# Autodesk Inventor assembly: UpperBody
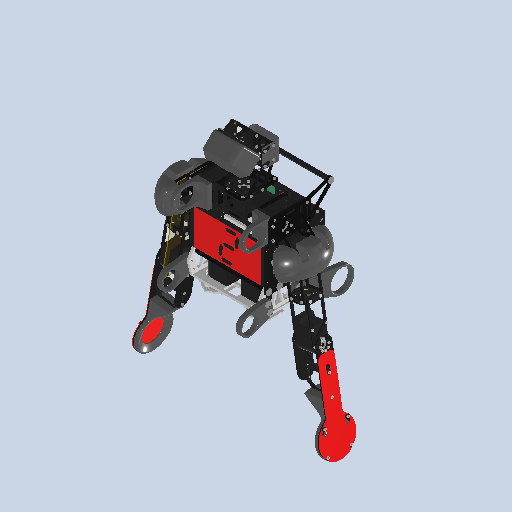
[picture p0: Inventor's stored thumbnail of the model, 512x512]
Saved by Autodesk Inventor 2022 (Build 260153000, 153)
## iProperties
Created: 2022-01-14
Part Number: UpperBody
Document SubType Name: Assembly
Designer: Masato Kubotera
Mass: 1918.95 g
Surface Area: 7006.93 cm^2
Volume: 1229.13 cm^3
Author: Masato Kubotera
## Documents named in this file (11)
- C:\Users\Masato\Documents\Inventor\CIT Brains_Inventor\SUSTAINA-OP\UpperBody\UpperBody.iam
- C:\Users\Masato\Documents\Inventor\CIT Brains_Inventor\SUSTAINA-OP\UpperBody\Trunk\Trunk.iam
- C:\Users\Masato\Documents\Inventor\CIT Brains_Inventor\SUSTAINA-OP\UpperBody\Head\Head.iam
- C:\Users\Masato\Documents\Inventor\CIT Brains_Inventor\SUSTAINA-OP\UpperBody\Arm\Shoulder.iam
- C:\Users\Masato\Documents\Inventor\CIT Brains_Inventor\SUSTAINA-OP\UpperBody\Arm\UpperArm.iam
- C:\Users\Masato\Documents\Inventor\CIT Brains_Inventor\SUSTAINA-OP\UpperBody\Arm\ForeArm.iam
- C:\Users\Masato\Documents\Inventor\CIT Brains_Inventor\SUSTAINA-OP\UpperBody\Arm\UpperArm_MIR.iam
- C:\Users\Masato\Documents\Inventor\CIT Brains_Inventor\SUSTAINA-OP\UpperBody\Cockpit\Cockpit.iam
- C:\Users\Masato\Documents\Inventor\CIT Brains_Inventor\SUSTAINA-OP\UpperBody\Arm\ForeArm_hand.ipt
- C:\Users\Masato\Documents\Inventor\CIT Brains_Inventor\SUSTAINA-OP\ReadyMade\InsertNut\UD-43040.ipt
- C:\Users\Masato\Documents\Inventor\CIT Brains_Inventor\SUSTAINA-OP\UpperBody\Arm\SideBumper.ipt
## Components (21 placed, 10 different names)
1. Trunk:1 [sub-assembly] — フラッシュ:1, フラッシュ:2, フラッシュ:3, 挿入:1, 角度:1, 挿入:2, 挿入:3, 角度:2, 角度:3, 挿入:11
2. Head:1 [sub-assembly] — 挿入:1, 角度:1
3. Shoulder:1 [sub-assembly] — 挿入:2, 角度:2, 挿入:4, 角度:4
4. Shoulder:2 [sub-assembly] — 挿入:3, 角度:3, 挿入:9, 角度:7
5. UpperArm:1 [sub-assembly] — 挿入:4, 角度:4, 挿入:6, 角度:6, フラッシュ:4, フラッシュ:5, フラッシュ:6
6. ForeArm:1 [sub-assembly] — 挿入:6, 角度:6, 挿入:20, 挿入:21
7. ForeArm:2 [sub-assembly] — 挿入:10, 角度:8, 挿入:22, 挿入:23
8. UpperArm_MIR:1 [sub-assembly] — 挿入:9, 挿入:10, 角度:7, 角度:8, メイト:1, メイト:2, フラッシュ:7
9. Cockpit:1 [sub-assembly] — 挿入:11, 角度:9
10. ForeArm_hand:1 — 挿入:12, 挿入:13, 挿入:14, 挿入:15
11. ForeArm_hand:2 — 挿入:16, 挿入:17, 挿入:18, 挿入:19
12. SideBumper:1 — フラッシュ:4, フラッシュ:5, フラッシュ:6
13. SideBumper:2 — メイト:1, メイト:2, フラッシュ:7
14. UD-43040:1 — 挿入:12, 挿入:20
15. UD-43040:2 — 挿入:13, 挿入:21
16. UD-43040:3 — 挿入:14
17. UD-43040:4 — 挿入:15
18. UD-43040:5 — 挿入:16, 挿入:23
19. UD-43040:6 — 挿入:17
20. UD-43040:7 — 挿入:18, 挿入:22
21. UD-43040:8 — 挿入:19
## Relationships (37: Insert 20, Angle 8, Flush 7, Mate 2)
- フラッシュ:1 [Flush]: Trunk:1
- フラッシュ:2 [Flush]: Trunk:1
- フラッシュ:3 [Flush]: Trunk:1
- 挿入:1 [Insert]: Trunk:1 ↔ Head:1
- 角度:1 [Angle] (0 deg): Trunk:1 ↔ Head:1
- 挿入:2 [Insert]: Trunk:1 ↔ Shoulder:1
- 挿入:3 [Insert]: Trunk:1 ↔ Shoulder:2
- 角度:2 [Angle] (0 deg): Trunk:1 ↔ Shoulder:1
- 角度:3 [Angle] (0 deg): Trunk:1 ↔ Shoulder:2
- 挿入:4 [Insert]: Shoulder:1 ↔ UpperArm:1
- 角度:4 [Angle] (170 deg): Shoulder:1 ↔ UpperArm:1
- 挿入:6 [Insert]: UpperArm:1 ↔ ForeArm:1
- 角度:6 [Angle] (0 deg): UpperArm:1 ↔ ForeArm:1
- 挿入:9 [Insert]: Shoulder:2 ↔ UpperArm_MIR:1
- 挿入:10 [Insert]: ForeArm:2 ↔ UpperArm_MIR:1
- 角度:7 [Angle] (10 deg): Shoulder:2 ↔ UpperArm_MIR:1
- 角度:8 [Angle] (180 deg): ForeArm:2 ↔ UpperArm_MIR:1
- 挿入:11 [Insert] (0.025 mm): Trunk:1 ↔ Cockpit:1
- 角度:9 [Angle] (0 deg): Cockpit:1
- 挿入:12 [Insert]: ForeArm_hand:1 ↔ UD-43040:1
- 挿入:13 [Insert]: ForeArm_hand:1 ↔ UD-43040:2
- 挿入:14 [Insert]: ForeArm_hand:1 ↔ UD-43040:3
- 挿入:15 [Insert]: ForeArm_hand:1 ↔ UD-43040:4
- 挿入:16 [Insert]: ForeArm_hand:2 ↔ UD-43040:5
- 挿入:17 [Insert]: ForeArm_hand:2 ↔ UD-43040:6
- 挿入:18 [Insert]: ForeArm_hand:2 ↔ UD-43040:7
- 挿入:19 [Insert]: ForeArm_hand:2 ↔ UD-43040:8
- 挿入:20 [Insert]: ForeArm:1 ↔ UD-43040:1
- 挿入:21 [Insert]: ForeArm:1 ↔ UD-43040:2
- 挿入:22 [Insert]: ForeArm:2 ↔ UD-43040:7
- 挿入:23 [Insert]: ForeArm:2 ↔ UD-43040:5
- フラッシュ:4 [Flush]: UpperArm:1 ↔ SideBumper:1
- フラッシュ:5 [Flush]: UpperArm:1 ↔ SideBumper:1
- フラッシュ:6 [Flush]: UpperArm:1 ↔ SideBumper:1
- メイト:1 [Mate]: UpperArm_MIR:1 ↔ SideBumper:2
- メイト:2 [Mate]: UpperArm_MIR:1 ↔ SideBumper:2
- フラッシュ:7 [Flush]: UpperArm_MIR:1 ↔ SideBumper:2
